# Autodesk Inventor assembly: ZLW-1040-OD-02-S-200-L_R-1200
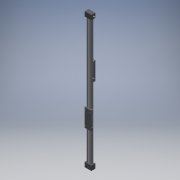
[picture p0: Inventor's stored thumbnail of the model, 180x180]
Saved by Autodesk Inventor 2019 (Build 230136000, 136)
## iProperties
Created: 2019-01-30
Part Number: ZLW-1040-OD-02-S-200-L_R-1200
Document SubType Name: Assembly
Designer: Michael Olukoya
Major Version: 0.0
Minor Version: 0.0
Format Version: 0.0
Author: Michael Olukoya
## Documents named in this file (4)
- C:\Users\Michael Olukoya\Desktop\Turtle BOT- AI\New Bot components\IGUS Rail\ZLW-1040-OD-02-S-200-L_R-1200.iam
- C:\Users\Michael Olukoya\Desktop\Turtle BOT- AI\New Bot components\IGUS Rail\ZLW-1040-OD-02-S-200-L_R-1200.ipt
- C:\Users\Michael Olukoya\Desktop\Turtle BOT- AI\New Bot components\IGUS Rail\ZLW-1040-OD-02-S-200-L_R-1200_1.ipt
- C:\Users\Michael Olukoya\Desktop\Turtle BOT- AI\New Bot components\IGUS Rail\ZLW-1040-OD-02-S-200-L_R-1200_2.ipt
## Components (3 placed, 3 different names)
1. ZLW-1040-OD-02-S-200-L_R-1200_1:1 — Mate:1, Mate:2, Mate:5
2. ZLW-1040-OD-02-S-200-L_R-1200_2:1 — Mate:3, Mate:4, Mate:6
3. ZLW-1040-OD-02-S-200-L_R-1200_3:1 — Mate:1, Mate:2, Mate:3, Mate:4, Mate:5, Mate:6
## Relationships (6: Mate 6)
- Mate:1: ZLW-1040-OD-02-S-200-L_R-1200_1:1 ↔ ZLW-1040-OD-02-S-200-L_R-1200_3:1
- Mate:2: ZLW-1040-OD-02-S-200-L_R-1200_1:1 ↔ ZLW-1040-OD-02-S-200-L_R-1200_3:1
- Mate:3: ZLW-1040-OD-02-S-200-L_R-1200_2:1 ↔ ZLW-1040-OD-02-S-200-L_R-1200_3:1
- Mate:4: ZLW-1040-OD-02-S-200-L_R-1200_2:1 ↔ ZLW-1040-OD-02-S-200-L_R-1200_3:1
- Mate:5: ZLW-1040-OD-02-S-200-L_R-1200_1:1 ↔ ZLW-1040-OD-02-S-200-L_R-1200_3:1
- Mate:6: ZLW-1040-OD-02-S-200-L_R-1200_2:1 ↔ ZLW-1040-OD-02-S-200-L_R-1200_3:1
